# Autodesk Inventor assembly: UNLHEP-14-A-01-007_Picker
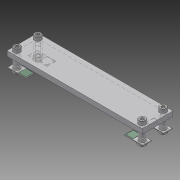
[picture p0: Inventor's stored thumbnail of the model, 180x180]
Saved by Autodesk Inventor 2013 (Build 170138000, 138)
## iProperties
Created: 2014-01-23
Part Number: UNLHEP-14-A-01-007_Picker
Document SubType Name: Assembly
Designer: Frank Meier
Project: UNL Pixel Phase I
Author: Frank Meier
## Documents named in this file (7)
- C:\Users\Frank Meier\Documents\Inventor\Delvotec-Saugplatte\UNLHEP-14-01-A-007_Picker.iam
- C:\Users\Frank Meier\Documents\Inventor\Delvotec-Saugplatte\UNLHEP-14-01-P-013_PickerPlate.ipt
- C:\Users\Frank Meier\Documents\Inventor\Content Center Files\R2013\de-DE\ISO 4762(2)\ISO 4762 - M3 x 16ISO.ipt
- C:\Users\Frank Meier\Documents\Inventor\Delvotec-Saugplatte\UNLHEP-14-01-P-014_PickerDistanceRing.ipt
- C:\Users\Frank Meier\Documents\Inventor\Delvotec-Saugplatte\UNLHEP-14-01-P-015_PickerStrip.ipt
- C:\Users\Frank Meier\Documents\Inventor\Content Center Files\R2013\de-DE\ISO 4032(1)\ISO 4032 - M3DIN EN.ipt
- C:\Users\Frank Meier\Documents\Inventor\Delvotec-Saugplatte\UNLHEP-14-01-P-018_PickerRubberPiece.ipt
## Components (21 placed, 6 different names)
1. UNLHEP-14-01-P-013_PickerPlate:1 — Einfügen:1, Einfügen:2, Einfügen:3, Einfügen:4, Passend:2, Passend:5, Passend:7, Passend:9
2. ISO 4762 M3 x 16:1 — Einfügen:1, Passend:6, Passend:12, Passend:17
3. ISO 4762 M3 x 16:2 — Einfügen:2, Passend:8, Passend:14, Passend:23
4. ISO 4762 M3 x 16:3 — Einfügen:3, Passend:10, Passend:16, Passend:21
5. ISO 4762 M3 x 16:4 — Einfügen:4, Passend:1, Passend:4, Passend:19
6. UNLHEP-14-01-P-014_PickerDistanceRing:1 — Passend:1, Passend:2, Passend:3
7. UNLHEP-14-01-P-015_PickerStrip:1 — Passend:3, Passend:4, Passend:20, Passend:28, Passend:29, Passend:30
8. UNLHEP-14-01-P-014_PickerDistanceRing:2 — Passend:5, Passend:6, Passend:11
9. UNLHEP-14-01-P-014_PickerDistanceRing:3 — Passend:7, Passend:8, Passend:13
10. UNLHEP-14-01-P-014_PickerDistanceRing:4 — Passend:9, Passend:10, Passend:15
11. UNLHEP-14-01-P-015_PickerStrip:2 — Passend:11, Passend:12, Passend:18, Passend:25, Passend:26, Passend:27
12. UNLHEP-14-01-P-015_PickerStrip:3 — Passend:15, Passend:16, Passend:22, Passend:31, Passend:35, Passend:36
13. UNLHEP-14-01-P-015_PickerStrip:4 — Passend:13, Passend:14, Passend:24, Passend:32, Passend:33, Passend:34
14. DIN EN 24032 M3:1 — Passend:17, Passend:18
15. DIN EN 24032 M3:2 — Passend:19, Passend:20
16. DIN EN 24032 M3:3 — Passend:21, Passend:22
17. DIN EN 24032 M3:4 — Passend:23, Passend:24
18. UNLHEP-14-01-P-018_PickerRubberPiece:1 — Passend:25, Passend:26, Passend:27
19. UNLHEP-14-01-P-018_PickerRubberPiece:2 — Passend:28, Passend:29, Passend:30
20. UNLHEP-14-01-P-018_PickerRubberPiece:3 — Passend:31, Passend:35, Passend:36
21. UNLHEP-14-01-P-018_PickerRubberPiece:4 — Passend:32, Passend:33, Passend:34
## Relationships (40: Mate 36, Insert 4)
- Passend:1 [Mate]: ISO 4762 M3 x 16:4 ↔ UNLHEP-14-01-P-014_PickerDistanceRing:1
- Passend:2 [Mate]: UNLHEP-14-01-P-013_PickerPlate:1 ↔ UNLHEP-14-01-P-014_PickerDistanceRing:1
- Passend:3 [Mate]: UNLHEP-14-01-P-014_PickerDistanceRing:1 ↔ UNLHEP-14-01-P-015_PickerStrip:1
- Passend:4 [Mate]: ISO 4762 M3 x 16:4 ↔ UNLHEP-14-01-P-015_PickerStrip:1
- Passend:5 [Mate]: UNLHEP-14-01-P-013_PickerPlate:1 ↔ UNLHEP-14-01-P-014_PickerDistanceRing:2
- Passend:6 [Mate]: ISO 4762 M3 x 16:1 ↔ UNLHEP-14-01-P-014_PickerDistanceRing:2
- Passend:7 [Mate]: UNLHEP-14-01-P-013_PickerPlate:1 ↔ UNLHEP-14-01-P-014_PickerDistanceRing:3
- Passend:8 [Mate]: ISO 4762 M3 x 16:2 ↔ UNLHEP-14-01-P-014_PickerDistanceRing:3
- Passend:9 [Mate]: UNLHEP-14-01-P-013_PickerPlate:1 ↔ UNLHEP-14-01-P-014_PickerDistanceRing:4
- Passend:10 [Mate]: ISO 4762 M3 x 16:3 ↔ UNLHEP-14-01-P-014_PickerDistanceRing:4
- Passend:11 [Mate]: UNLHEP-14-01-P-014_PickerDistanceRing:2 ↔ UNLHEP-14-01-P-015_PickerStrip:2
- Passend:12 [Mate]: ISO 4762 M3 x 16:1 ↔ UNLHEP-14-01-P-015_PickerStrip:2
- Passend:13 [Mate]: UNLHEP-14-01-P-014_PickerDistanceRing:3 ↔ UNLHEP-14-01-P-015_PickerStrip:4
- Passend:14 [Mate]: ISO 4762 M3 x 16:2 ↔ UNLHEP-14-01-P-015_PickerStrip:4
- Passend:15 [Mate]: UNLHEP-14-01-P-014_PickerDistanceRing:4 ↔ UNLHEP-14-01-P-015_PickerStrip:3
- Passend:16 [Mate]: ISO 4762 M3 x 16:3 ↔ UNLHEP-14-01-P-015_PickerStrip:3
- Passend:18 [Mate]: UNLHEP-14-01-P-015_PickerStrip:2 ↔ DIN EN 24032 M3:1
- Passend:20 [Mate]: UNLHEP-14-01-P-015_PickerStrip:1 ↔ DIN EN 24032 M3:2
- Passend:22 [Mate]: UNLHEP-14-01-P-015_PickerStrip:3 ↔ DIN EN 24032 M3:3
- Passend:24 [Mate]: UNLHEP-14-01-P-015_PickerStrip:4 ↔ DIN EN 24032 M3:4
- Passend:25 [Mate]: UNLHEP-14-01-P-015_PickerStrip:2 ↔ UNLHEP-14-01-P-018_PickerRubberPiece:1
- Passend:26 [Mate] (0.5 mm): UNLHEP-14-01-P-015_PickerStrip:2 ↔ UNLHEP-14-01-P-018_PickerRubberPiece:1
- Passend:27 [Mate] (0.5 mm): UNLHEP-14-01-P-015_PickerStrip:2 ↔ UNLHEP-14-01-P-018_PickerRubberPiece:1
- Passend:28 [Mate]: UNLHEP-14-01-P-015_PickerStrip:1 ↔ UNLHEP-14-01-P-018_PickerRubberPiece:2
- Passend:29 [Mate] (0.5 mm): UNLHEP-14-01-P-015_PickerStrip:1 ↔ UNLHEP-14-01-P-018_PickerRubberPiece:2
- Passend:30 [Mate] (0.5 mm): UNLHEP-14-01-P-015_PickerStrip:1 ↔ UNLHEP-14-01-P-018_PickerRubberPiece:2
- Passend:31 [Mate]: UNLHEP-14-01-P-015_PickerStrip:3 ↔ UNLHEP-14-01-P-018_PickerRubberPiece:3
- Passend:32 [Mate]: UNLHEP-14-01-P-015_PickerStrip:4 ↔ UNLHEP-14-01-P-018_PickerRubberPiece:4
- Passend:33 [Mate] (0.5 mm): UNLHEP-14-01-P-015_PickerStrip:4 ↔ UNLHEP-14-01-P-018_PickerRubberPiece:4
- Passend:34 [Mate] (0.5 mm): UNLHEP-14-01-P-015_PickerStrip:4 ↔ UNLHEP-14-01-P-018_PickerRubberPiece:4
- Passend:35 [Mate] (0.5 mm): UNLHEP-14-01-P-015_PickerStrip:3 ↔ UNLHEP-14-01-P-018_PickerRubberPiece:3
- Passend:36 [Mate] (0.5 mm): UNLHEP-14-01-P-015_PickerStrip:3 ↔ UNLHEP-14-01-P-018_PickerRubberPiece:3
- Einfügen:1 [Insert]: UNLHEP-14-01-P-013_PickerPlate:1 ↔ ISO 4762 M3 x 16:1
- Einfügen:2 [Insert]: UNLHEP-14-01-P-013_PickerPlate:1 ↔ ISO 4762 M3 x 16:2
- Einfügen:3 [Insert]: UNLHEP-14-01-P-013_PickerPlate:1 ↔ ISO 4762 M3 x 16:3
- Einfügen:4 [Insert]: UNLHEP-14-01-P-013_PickerPlate:1 ↔ ISO 4762 M3 x 16:4
- Passend:17 [Mate]: ISO 4762 M3 x 16:1 ↔ DIN EN 24032 M3:1
- Passend:19 [Mate]: ISO 4762 M3 x 16:4 ↔ DIN EN 24032 M3:2
- Passend:21 [Mate]: ISO 4762 M3 x 16:3 ↔ DIN EN 24032 M3:3
- Passend:23 [Mate]: ISO 4762 M3 x 16:2 ↔ DIN EN 24032 M3:4
